# Autodesk Inventor assembly: Assy_flame_side_left
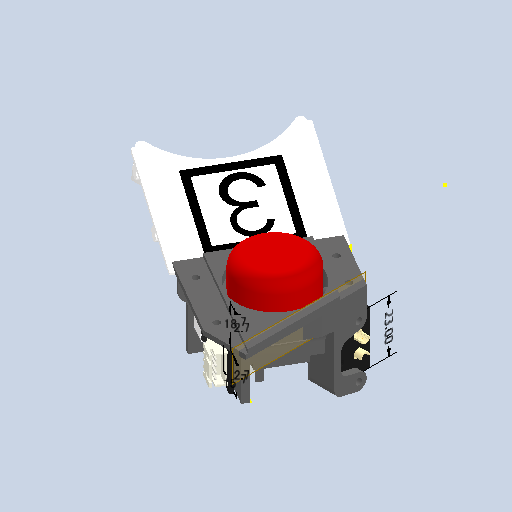
[picture p0: Inventor's stored thumbnail of the model, 512x512]
Saved by Autodesk Inventor 2024.1 (Build 281209000, 209)
## iProperties
Created: 2025-05-04
Part Number: Assy_flame_side_left
Document SubType Name: Assembly
Designer: hibik
Author: hibik
## Documents named in this file (6)
- C:\Users\hibik\Documents\Robomech\RESCUE\ORCA\hard\flame_back\Assy_flame_side_left.iam
- C:\Users\hibik\Documents\Robomech\RESCUE\ORCA\hard\flame_back\flame_side_left.ipt
- C:\Users\hibik\Documents\Robomech\RESCUE\ORCA\hard\std_parts\emergency_button.ipt
- C:\Users\hibik\Documents\Robomech\RESCUE\ORCA\hard\cover\cover_side.ipt
- C:\Users\hibik\Documents\Robomech\RESCUE\ORCA\hard\board\CORE_model\external_io_external_input.iam
- C:\Users\hibik\Documents\Robomech\RESCUE\ORCA\hard\board\CORE_model\type_c.iam
## Components (5 placed, 5 different names)
1. flame_side_left:1 — 挿入:1, 角度:1, 挿入:2, 挿入:3, 角度:2, 角度:3, フラッシュ:1, 挿入:4, 角度:4
2. emergency_button:1 — 挿入:1, 角度:1
3. cover_side:1 — 挿入:2
4. external_io_external_input:1 [sub-assembly] — 挿入:3, 角度:2, フラッシュ:1
5. type_c:1 [sub-assembly] — 角度:3, 挿入:4, 角度:4
## Relationships (9: Insert 4, Angle 4, Flush 1)
- 挿入:1 [Insert]: flame_side_left:1 ↔ emergency_button:1
- 角度:1 [Angle] (0 deg): flame_side_left:1 ↔ emergency_button:1
- 挿入:2 [Insert] (0.25 mm): flame_side_left:1 ↔ cover_side:1
- 挿入:3 [Insert]: flame_side_left:1 ↔ external_io_external_input:1
- 角度:2 [Angle] (0 deg): flame_side_left:1 ↔ external_io_external_input:1
- 角度:3 [Angle] (0 deg): flame_side_left:1 ↔ type_c:1
- フラッシュ:1 [Flush]: flame_side_left:1 ↔ external_io_external_input:1
- 挿入:4 [Insert]: flame_side_left:1 ↔ type_c:1
- 角度:4 [Angle] (0 deg): flame_side_left:1 ↔ type_c:1
